# Autodesk Inventor assembly: BAssembly1
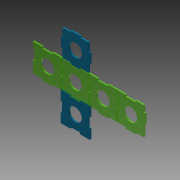
[picture p0: Inventor's stored thumbnail of the model, 180x180]
Saved by Autodesk Inventor 2014 SP2 (Build 180246200, 246)
## iProperties
Created: 2014-11-24
Part Number: BAssembly1
Document SubType Name: Assembly
Designer: JLM
Author: JLM
## Documents named in this file (4)
- C:\Users\JLM\Documents\Art\Puzzle Box\BSizeBox\BAssembly1.iam
- C:\Users\JLM\Documents\Art\Puzzle Box\BSizeBox\BBottom.ipt
- C:\Users\JLM\Documents\Art\Puzzle Box\BSizeBox\BSide.ipt
- C:\Users\JLM\Documents\Art\Puzzle Box\BSizeBox\BTop.ipt
## Components (6 placed, 3 different names)
1. BBottom:1 — Mate:3, Flush:8, Mate:4
2. BTop:2 — Mate:8
3. BSide:3 — Mate:3, Flush:8, Flush:9, Flush:10, Flush:12, Flush:14, Mate:4, Mate:5, Mate:6, Mate:8
4. BSide:4 — Flush:10, Flush:11, Flush:13, Flush:14, Mate:6, Mate:7
5. BSide:5 — Flush:9, Flush:12, Mate:5
6. BSide:6 — Flush:11, Flush:13, Mate:7
## Relationships (13: Flush 7, Mate 6)
- Mate:3: BBottom:1 ↔ BSide:3
- Flush:8: BBottom:1 ↔ BSide:3
- Flush:9: BSide:3 ↔ BSide:5
- Flush:10: BSide:3 ↔ BSide:4
- Flush:11: BSide:4 ↔ BSide:6
- Flush:12: BSide:3 ↔ BSide:5
- Flush:13: BSide:4 ↔ BSide:6
- Flush:14: BSide:3 ↔ BSide:4
- Mate:4: BBottom:1 ↔ BSide:3
- Mate:5: BSide:3 ↔ BSide:5
- Mate:6: BSide:3 ↔ BSide:4
- Mate:7: BSide:4 ↔ BSide:6
- Mate:8: BTop:2 ↔ BSide:3
